# Autodesk Inventor assembly: ServoLegAssembly
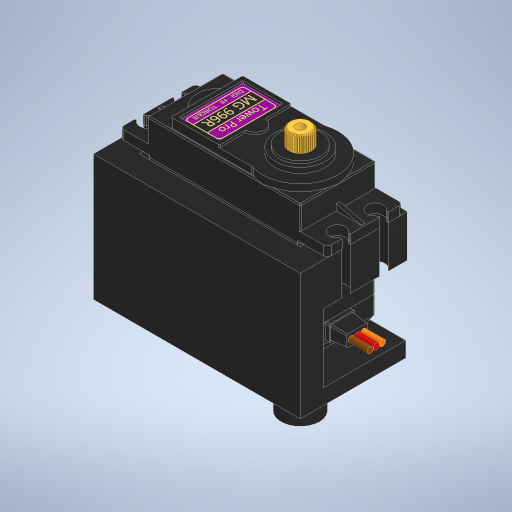
[picture p0: Inventor's stored thumbnail of the model, 512x512]
Saved by Autodesk Inventor 2024 (Build 280153000, 153)
## iProperties
Created: 2024-09-07
Part Number: ServoLegAssembly
Document SubType Name: Assembly
Designer: omiye
Author: omiye
## Documents named in this file (3)
- C:\Projects\Arduino\hexapod\legModels\stls\ServoLegAssembly.iam
- C:\Projects\Arduino\hexapod\legModels\MG996RServo.ipt
- C:\Projects\Arduino\hexapod\legModels\MG996RServoHolder.ipt
## Components (2 placed, 2 different names)
1. MG996RServo:1 — Mate:1, Mate:2
2. MG996RServoHolder:1 — Mate:1, Mate:2
## Relationships (2: Mate 2)
- Mate:1: MG996RServo:1 ↔ MG996RServoHolder:1
- Mate:2: MG996RServo:1 ↔ MG996RServoHolder:1
